# Autodesk Inventor assembly: Cup_Dispenser
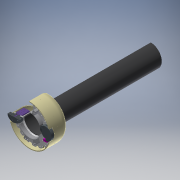
[picture p0: Inventor's stored thumbnail of the model, 180x180]
Saved by Autodesk Inventor 2016 (Build 200138000, 138)
## iProperties
Created: 2015-07-19
Part Number: Cup_Dispenser
Document SubType Name: Assembly
Designer: bastli
Author: bastli
## Documents named in this file (9)
- C:\Users\3DPrinterUser\Documents\GitHub\BarBot\Conception\Mechanical\Cup_Dispenser_3\Cup_Dispenser.iam
- C:\Users\3DPrinterUser\Documents\GitHub\BarBot\Conception\Mechanical\Cup_Dispenser_3\Fixture.ipt
- C:\Users\3DPrinterUser\Documents\GitHub\BarBot\Conception\Mechanical\Cup_Dispenser_3\Transmission.ipt
- C:\Users\3DPrinterUser\Documents\GitHub\BarBot\Conception\Mechanical\Cup_Dispenser_3\Nema 8.ipt
- C:\Users\3DPrinterUser\Documents\GitHub\BarBot\Conception\Mechanical\Cup_Dispenser_3\Funnel_Adapter.ipt
- C:\Users\3DPrinterUser\Documents\GitHub\BarBot\Conception\Mechanical\Cup_Dispenser_3\Hull.ipt
- C:\Users\3DPrinterUser\Documents\GitHub\BarBot\Conception\Mechanical\Cup_Dispenser\Cup_Dispenser_Pipe.ipt
- C:\Users\3DPrinterUser\Documents\GitHub\BarBot\Conception\Mechanical\Cup_Dispenser_3\Board_Shape.ipt
- C:\Users\3DPrinterUser\Documents\GitHub\BarBot\Conception\Mechanical\Cup_Dispenser_3\Microswitch_Fixture.ipt
## Components (13 placed, 8 different names)
1. Fixture:1 — Rigid:1, Rigid:3, Flush:1, Flush:2, Rigid:4, Flush:3, Rotational:4, Rotational:5, Flush:4, Rigid:5
2. Transmission:1 — Rotational:1
3. Nema 8:1 — Rigid:1, Rotational:1
4. Nema 8:2 — Rigid:3, Rotational:2
5. Transmission:2 — Rotational:2
6. Funnel_Adapter:1 — Flush:1
7. Hull:1 — Flush:2
8. Cup_Dispenser_Pipe:1 — Rigid:4
9. Board_Shape:1 — Flush:3
10. Board_Shape:2 — Rotational:4
11. Funnel_Adapter:2 — Rotational:5
12. Microswitch_Fixture:1 — Flush:4
13. Microswitch_Fixture:2 — Rigid:5
## Relationships (12: WeldJoint 4, RevoluteJoint 4, Flush 4)
- Rigid:1 [WeldJoint]: Fixture:1 ↔ Nema 8:1
- Rotational:1 [RevoluteJoint]: Transmission:1 ↔ Nema 8:1
- Rigid:3 [WeldJoint]: Fixture:1 ↔ Nema 8:2
- Rotational:2 [RevoluteJoint]: Nema 8:2 ↔ Transmission:2
- Flush:1: Fixture:1 ↔ Funnel_Adapter:1
- Flush:2: Fixture:1 ↔ Hull:1
- Rigid:4 [WeldJoint]: Fixture:1 ↔ Cup_Dispenser_Pipe:1
- Flush:3: Fixture:1 ↔ Board_Shape:1
- Rotational:4 [RevoluteJoint]: Fixture:1 ↔ Board_Shape:2
- Rotational:5 [RevoluteJoint]: Fixture:1 ↔ Funnel_Adapter:2
- Flush:4: Fixture:1 ↔ Microswitch_Fixture:1
- Rigid:5 [WeldJoint]: Fixture:1 ↔ Microswitch_Fixture:2
